# Autodesk Inventor assembly: Neck Support
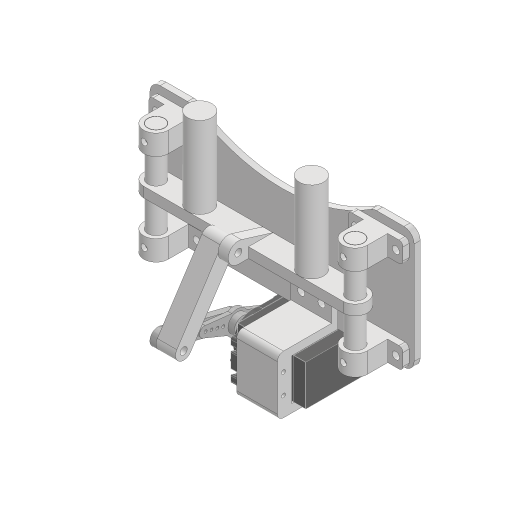
[picture p0: Inventor's stored thumbnail of the model, 512x512]
Saved by Autodesk Inventor 2024 (Build 280153000, 153)
## iProperties
Created: 2025-04-26
Part Number: Neck Support
Document SubType Name: Assembly
Designer: Binara
Author: Binara
## Documents named in this file (10)
- Z:\Robotics\Inventor\Auto Chair\Neck Support\Neck Support.iam
- Z:\Robotics\Inventor\Auto Chair\Neck Support\Base plate.ipt
- Z:\Robotics\Inventor\Auto Chair\Neck Support\Rod Holder.ipt
- Z:\Robotics\Inventor\Auto Chair\Neck Support\Neck support rod.ipt
- Z:\Robotics\Inventor\Auto Chair\Neck Support\Support slider.ipt
- Z:\Robotics\Inventor\Auto Chair\Auto Chair\Mg995 v1.ipt
- Z:\Robotics\Inventor\Auto Chair\Auto Chair\MG995_Gear2 v1.ipt
- Z:\Robotics\Inventor\Auto Chair\Neck Support\Servo mount.ipt
- Z:\Robotics\Inventor\Auto Chair\Auto Chair\Servo Small Arm.ipt
- Z:\Robotics\Inventor\Auto Chair\Neck Support\Neck Servo Arm.ipt
## Components (13 placed, 9 different names)
1. Base plate:1 — Mate:1, Rigid:2, Rigid:1, Rigid:3, Rigid:4, Mate:4, Angle:1
2. Rod Holder:1 — Mate:1, Rigid:2, Rotational:2
3. Rod Holder:2 — Rigid:1
4. Rod Holder:3 — Rigid:3
5. Rod Holder:4 — Rigid:4, Rotational:1
6. Neck support rod:1 — Rotational:1, Mate:3
7. Neck support rod:2 — Rotational:2, Mate:2
8. Support slider:1 — Mate:2, Mate:3, Rotational:6
9. Mg995 v1:1 — Mate:4, Angle:1, Rotational:3, Rotational:4
10. MG995_Gear2 v1:1 — Rotational:3, Rotational:5, Mate:5
11. Servo mount:1 — Rotational:4
12. Servo Small Arm:1 — Rotational:5, Mate:5, Mate:6
13. Neck Servo Arm:1 — Rotational:6, Mate:6
## Relationships (17: Mate 6, RevoluteJoint 6, WeldJoint 4, Angle 1)
- Mate:1: Base plate:1 ↔ Rod Holder:1
- Rigid:2 [WeldJoint]: Base plate:1 ↔ Rod Holder:1
- Rigid:1 [WeldJoint]: Base plate:1 ↔ Rod Holder:2
- Rigid:3 [WeldJoint]: Base plate:1 ↔ Rod Holder:3
- Rigid:4 [WeldJoint]: Base plate:1 ↔ Rod Holder:4
- Rotational:1 [RevoluteJoint]: Rod Holder:4 ↔ Neck support rod:1
- Rotational:2 [RevoluteJoint]: Rod Holder:1 ↔ Neck support rod:2
- Mate:2: Neck support rod:2 ↔ Support slider:1
- Mate:3: Neck support rod:1 ↔ Support slider:1
- Mate:4: Base plate:1 ↔ Mg995 v1:1
- Angle:1 (0 deg): Base plate:1 ↔ Mg995 v1:1
- Rotational:3 [RevoluteJoint]: Mg995 v1:1 ↔ MG995_Gear2 v1:1
- Rotational:4 [RevoluteJoint]: Mg995 v1:1 ↔ Servo mount:1
- Rotational:5 [RevoluteJoint]: MG995_Gear2 v1:1 ↔ Servo Small Arm:1
- Mate:5: MG995_Gear2 v1:1 ↔ Servo Small Arm:1
- Rotational:6 [RevoluteJoint]: Support slider:1 ↔ Neck Servo Arm:1
- Mate:6: Servo Small Arm:1 ↔ Neck Servo Arm:1
